# Autodesk Inventor assembly: Assembly1
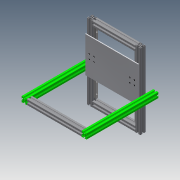
[picture p0: Inventor's stored thumbnail of the model, 180x180]
Saved by Autodesk Inventor 2016 (Build 200138000, 138)
## iProperties
Created: 2017-05-10
Part Number: Assembly1
Document SubType Name: Assembly
Designer: Spark Electronics
Author: Spark Electronics
## Documents named in this file (10)
- C:\Users\Owner\Documents\REZ_RAP\Assembly1.iam
- C:\Users\Owner\Documents\REZ_RAP\Y_CARRIAGE.ipt
- C:\Users\Owner\Documents\REZ_RAP\Y_carriage_90_bearing_mount.ipt
- C:\Users\Owner\Documents\REZ_RAP\15mm_bearing_rail_carriage.ipt
- C:\Users\Owner\Documents\REZ_RAP\y_Carriage_flat_head_8mm.ipt
- C:\Users\Owner\Documents\REZ_RAP\Y_carriage_bearing_rail.ipt
- C:\Users\Owner\Documents\REZ_RAP\Aluminum_extrusion.ipt
- C:\Users\Owner\Documents\REZ_RAP\ALuminum_extrusion_short.ipt
- C:\Users\Owner\Documents\REZ_RAP\Aluminum_extrusion_Z.ipt
- C:\Users\Owner\Documents\REZ_RAP\Aluminum_extrusion_Z_top.ipt
## Components (22 placed, 9 different names)
1. Y_CARRIAGE:1 — Mate:9, Mate:10
2. y_Carriage_flat_head_8mm:1
3. y_Carriage_flat_head_8mm:2
4. y_Carriage_flat_head_8mm:3
5. y_Carriage_flat_head_8mm:4
6. y_Carriage_flat_head_8mm:5
7. y_Carriage_flat_head_8mm:6
8. y_Carriage_flat_head_8mm:7
9. y_Carriage_flat_head_8mm:8
10. Y_carriage_90_bearing_mount:1 — Mate:9, Mate:12, Mate:15, Mate:16
11. Y_carriage_90_bearing_mount:2 — Mate:10, Mate:11, Mate:13, Mate:14
12. 15mm_bearing_rail_carriage:1 — Mate:12, Mate:15, Mate:16, Mate:20, Mate:22, Mate:25, Mate:26
13. 15mm_bearing_rail_carriage:2 — Mate:11, Mate:13, Mate:14, Mate:19, Mate:21, Mate:23, Mate:24
14. Y_carriage_bearing_rail:1 — Mate:19, Mate:21, Mate:23, Mate:24, Flush:11, Mate:30
15. Y_carriage_bearing_rail:2 — Mate:20, Mate:22, Mate:25, Mate:26, Flush:11, Mate:31, Mate:32, Flush:24
16. Aluminum_extrusion:1 — Flush:17, Flush:18, Flush:20, Flush:21, Mate:31, Flush:24, Mate:33, Mate:35, Flush:26, Mate:37, Flush:27
17. Aluminum_extrusion:2 — Flush:16, Flush:19, Flush:22, Flush:23, Mate:30, Mate:34, Flush:25, Mate:36, Flush:28
18. ALuminum_extrusion_short:1 — Flush:16, Flush:17, Flush:18, Flush:19, Flush:20, Mate:32, Mate:33, Mate:34
19. ALuminum_extrusion_short:2 — Flush:21, Flush:22, Flush:23, Mate:35
20. Aluminum_extrusion_Z:1 — Flush:25, Mate:36, Flush:28
21. Aluminum_extrusion_Z:2 — Flush:26, Mate:37, Flush:27, Mate:38, Flush:29, Flush:30
22. Aluminum_extrusion_Z_top:1 — Mate:38, Flush:29, Flush:30
## Relationships (59: Mate 35, Flush 24)
- [Mate]: Y_CARRIAGE:1 ↔ y_Carriage_flat_head_8mm:1
- [Mate]: Y_CARRIAGE:1 ↔ y_Carriage_flat_head_8mm:2
- [Mate]: Y_CARRIAGE:1 ↔ y_Carriage_flat_head_8mm:3
- [Mate]: Y_CARRIAGE:1 ↔ y_Carriage_flat_head_8mm:4
- [Mate]: Y_CARRIAGE:1 ↔ y_Carriage_flat_head_8mm:8
- [Mate]: Y_CARRIAGE:1 ↔ y_Carriage_flat_head_8mm:7
- [Mate]: Y_CARRIAGE:1 ↔ y_Carriage_flat_head_8mm:5
- [Mate]: Y_CARRIAGE:1 ↔ y_Carriage_flat_head_8mm:6
- [Flush]: Y_CARRIAGE:1 ↔ y_Carriage_flat_head_8mm:1
- [Flush]: Y_CARRIAGE:1 ↔ y_Carriage_flat_head_8mm:2
- [Flush]: Y_CARRIAGE:1 ↔ y_Carriage_flat_head_8mm:3
- [Flush]: Y_CARRIAGE:1 ↔ y_Carriage_flat_head_8mm:4
- [Flush]: Y_CARRIAGE:1 ↔ y_Carriage_flat_head_8mm:6
- [Flush]: Y_CARRIAGE:1 ↔ y_Carriage_flat_head_8mm:5
- [Flush]: Y_CARRIAGE:1 ↔ y_Carriage_flat_head_8mm:8
- [Flush]: Y_CARRIAGE:1 ↔ y_Carriage_flat_head_8mm:7
- Mate:9: Y_CARRIAGE:1 ↔ Y_carriage_90_bearing_mount:1
- Mate:10: Y_CARRIAGE:1 ↔ Y_carriage_90_bearing_mount:2
- Mate:11: Y_carriage_90_bearing_mount:2 ↔ 15mm_bearing_rail_carriage:2
- Mate:12: Y_carriage_90_bearing_mount:1 ↔ 15mm_bearing_rail_carriage:1
- Mate:13: Y_carriage_90_bearing_mount:2 ↔ 15mm_bearing_rail_carriage:2
- Mate:14: Y_carriage_90_bearing_mount:2 ↔ 15mm_bearing_rail_carriage:2
- Mate:15: Y_carriage_90_bearing_mount:1 ↔ 15mm_bearing_rail_carriage:1
- Mate:16: Y_carriage_90_bearing_mount:1 ↔ 15mm_bearing_rail_carriage:1
- [Mate]: y_Carriage_flat_head_8mm:5 ↔ Y_carriage_90_bearing_mount:2
- [Mate]: y_Carriage_flat_head_8mm:1 ↔ Y_carriage_90_bearing_mount:1
- Mate:19: 15mm_bearing_rail_carriage:2 ↔ Y_carriage_bearing_rail:1
- Mate:20: 15mm_bearing_rail_carriage:1 ↔ Y_carriage_bearing_rail:2
- Mate:21: 15mm_bearing_rail_carriage:2 ↔ Y_carriage_bearing_rail:1
- Mate:22: 15mm_bearing_rail_carriage:1 ↔ Y_carriage_bearing_rail:2
- Mate:23: 15mm_bearing_rail_carriage:2 ↔ Y_carriage_bearing_rail:1
- Mate:24: 15mm_bearing_rail_carriage:2 ↔ Y_carriage_bearing_rail:1
- Mate:25: 15mm_bearing_rail_carriage:1 ↔ Y_carriage_bearing_rail:2
- Mate:26: 15mm_bearing_rail_carriage:1 ↔ Y_carriage_bearing_rail:2
- Flush:11: Y_carriage_bearing_rail:1 ↔ Y_carriage_bearing_rail:2
- Flush:16: Aluminum_extrusion:2 ↔ ALuminum_extrusion_short:1
- Flush:17: Aluminum_extrusion:1 ↔ ALuminum_extrusion_short:1
- Flush:18: Aluminum_extrusion:1 ↔ ALuminum_extrusion_short:1
- Flush:19: Aluminum_extrusion:2 ↔ ALuminum_extrusion_short:1
- Flush:20: Aluminum_extrusion:1 ↔ ALuminum_extrusion_short:1
- Flush:21: Aluminum_extrusion:1 ↔ ALuminum_extrusion_short:2
- Flush:22: Aluminum_extrusion:2 ↔ ALuminum_extrusion_short:2
- Flush:23: Aluminum_extrusion:2 ↔ ALuminum_extrusion_short:2
- Mate:30 (-4 mm): Y_carriage_bearing_rail:1 ↔ Aluminum_extrusion:2
- Mate:31 (-4 mm): Y_carriage_bearing_rail:2 ↔ Aluminum_extrusion:1
- Mate:32 (12.7 mm): Y_carriage_bearing_rail:2 ↔ ALuminum_extrusion_short:1
- Flush:24 (-7.62 mm): Y_carriage_bearing_rail:2 ↔ Aluminum_extrusion:1
- Mate:33: Aluminum_extrusion:1 ↔ ALuminum_extrusion_short:1
- Mate:34: Aluminum_extrusion:2 ↔ ALuminum_extrusion_short:1
- Mate:35: Aluminum_extrusion:1 ↔ ALuminum_extrusion_short:2
- Flush:25 (228.6 mm): Aluminum_extrusion:2 ↔ Aluminum_extrusion_Z:1
- Flush:26 (228.6 mm): Aluminum_extrusion:1 ↔ Aluminum_extrusion_Z:2
- Mate:36 (3 mm): Aluminum_extrusion:2 ↔ Aluminum_extrusion_Z:1
- Mate:37 (3 mm): Aluminum_extrusion:1 ↔ Aluminum_extrusion_Z:2
- Flush:27 (-38.1 mm): Aluminum_extrusion:1 ↔ Aluminum_extrusion_Z:2
- Flush:28 (-38.1 mm): Aluminum_extrusion:2 ↔ Aluminum_extrusion_Z:1
- Mate:38: Aluminum_extrusion_Z:2 ↔ Aluminum_extrusion_Z_top:1
- Flush:29: Aluminum_extrusion_Z:2 ↔ Aluminum_extrusion_Z_top:1
- Flush:30: Aluminum_extrusion_Z:2 ↔ Aluminum_extrusion_Z_top:1
